# Autodesk Inventor assembly: arm
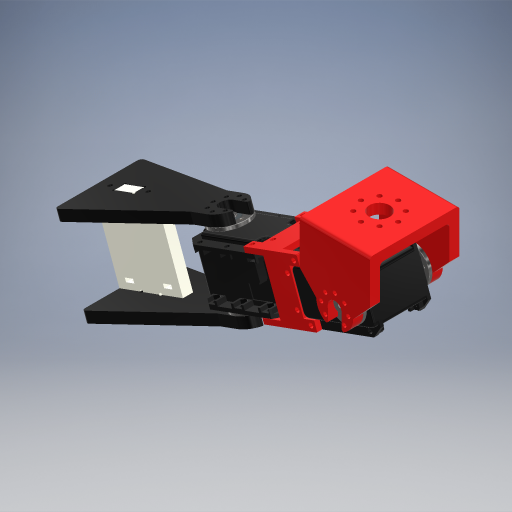
[picture p0: Inventor's stored thumbnail of the model, 512x512]
Saved by Autodesk Inventor 2024 (Build 280153000, 153)
## iProperties
Created: 2024-09-15
Part Number: arm
Document SubType Name: Assembly
Designer: msi
Author: msi
## Documents named in this file (8)
- C:\Users\msi\GITHUB\19th_intern_kgh_fight_robot\부품\Upper_body\Arm\arm_left.iam
- C:\Users\msi\GITHUB\19th_intern_kgh_fight_robot\부품\Upper_body\Arm\shoulder.ipt
- C:\Users\msi\GITHUB\19th_intern_kgh_fight_robot\부품\Upper_body\Arm\hand.ipt
- C:\Users\msi\GITHUB\19th_intern_kgh_fight_robot\부품\Upper_body\Arm\hand connection.ipt
- C:\Users\msi\GITHUB\19th_intern_kgh_fight_robot\부품\Upper_body\Arm\arm connection.ipt
- C:\Users\msi\GITHUB\19th_intern_kgh_fight_robot\부품\ROBOTIS(Inventor 2024 ver.)\다이나믹셀\MX-28T_R+idle.ipt.iam
- C:\Users\msi\GITHUB\19th_intern_kgh_fight_robot\부품\ROBOTIS(Inventor 2024 ver.)\혼\28Horn.ipt
- MX-28T_R+idle.ipt
## Components (9 placed, 6 different names)
1. shoulder:1 — 삽입:2, 삽입:3, 삽입:9, 각도:2
2. hand connection:1 — 삽입:12, 삽입:13, 삽입:14, 삽입:16
3. arm connection:1 — 삽입:4, 삽입:5, 삽입:7, 삽입:8, 각도:1
4. MX-28T_R+idle.ipt:1 [sub-assembly] — 삽입:1, 삽입:4, 삽입:5, 삽입:9, 각도:2
5. 28Horn:1 — 삽입:1, 삽입:2, 삽입:3
6. MX-28T_R+idle.ipt:2 [sub-assembly] — 삽입:7, 삽입:8, 삽입:15
7. 28Horn:2 — 삽입:10, 삽입:11
8. hand:2 — 삽입:10, 삽입:11, 삽입:12, 삽입:16, 각도:1
9. hand:3 — 삽입:13, 삽입:14, 삽입:15
## Relationships (18: Insert 16, Angle 2)
- 삽입:1 [Insert]: MX-28T_R+idle.ipt:1 ↔ 28Horn:1
- 삽입:2 [Insert]: shoulder:1 ↔ 28Horn:1
- 삽입:3 [Insert]: shoulder:1 ↔ 28Horn:1
- 삽입:4 [Insert]: arm connection:1 ↔ MX-28T_R+idle.ipt:1
- 삽입:5 [Insert]: arm connection:1 ↔ MX-28T_R+idle.ipt:1
- [Insert]: MX-28T_R+idle.ipt:2 ↔ 28Horn:2
- 삽입:7 [Insert]: arm connection:1 ↔ MX-28T_R+idle.ipt:2
- 삽입:8 [Insert]: arm connection:1 ↔ MX-28T_R+idle.ipt:2
- 삽입:9 [Insert]: shoulder:1 ↔ MX-28T_R+idle.ipt:1
- 삽입:10 [Insert]: 28Horn:2 ↔ hand:2
- 삽입:11 [Insert]: 28Horn:2 ↔ hand:2
- 삽입:12 [Insert]: hand connection:1 ↔ hand:2
- 삽입:13 [Insert]: hand connection:1 ↔ hand:3
- 삽입:14 [Insert]: hand connection:1 ↔ hand:3
- 삽입:15 [Insert]: MX-28T_R+idle.ipt:2 ↔ hand:3
- 삽입:16 [Insert]: hand connection:1 ↔ hand:2
- 각도:1 [Angle] (0 deg): arm connection:1 ↔ hand:2
- 각도:2 [Angle] (70 deg): shoulder:1 ↔ MX-28T_R+idle.ipt:1
## Named parameters: d5_d0 = 0 mm
